# Autodesk Inventor assembly: Drive Roller Assembly 3 (Lexan)
(part 2 of 2)
- Mate:1223: Vex Pro End Bearing Mount (Bolt):1 ↔ Bearing Mount Spacer 1-8 in:1
- Mate:1224: Vex Pro 1x1 rectangular tubing 14 in length:5 ↔ Bearing Mount Spacer 1-8 in:2
- Mate:1225: Vex Pro 1x1 rectangular tubing 14 in length:5 ↔ Bearing Mount Spacer 1-8 in:2
- Mate:1226: Vex Pro 1x1 rectangular tubing 14 in length:5 ↔ Bearing Mount Spacer 1-8 in:2
- Mate:1227: Vex Pro End Bearing Mount (Bolt):2 ↔ Bearing Mount Spacer 1-8 in:2
- Mate:1228: Vex Pro End Bearing Mount (Bolt):2 ↔ Bearing Mount Spacer 1-8 in:2
- Mate:1229: Vex Pro End Bearing Mount (Bolt):2 ↔ Bearing Mount Spacer 1-8 in:2
- Mate:1230: Vex Pro 1x1 rectangular tubing 14 in length:6 ↔ Bearing Mount Spacer 1-8 in:3
- Mate:1231: Vex Pro 1x1 rectangular tubing 14 in length:6 ↔ Bearing Mount Spacer 1-8 in:3
- Mate:1232: Vex Pro 1x1 rectangular tubing 14 in length:6 ↔ Bearing Mount Spacer 1-8 in:3
- Mate:1233: Vex Pro End Bearing Mount (Bolt):3 ↔ Bearing Mount Spacer 1-8 in:3
- Mate:1234: Vex Pro End Bearing Mount (Bolt):3 ↔ Bearing Mount Spacer 1-8 in:3
- Mate:1235: Vex Pro End Bearing Mount (Bolt):3 ↔ Bearing Mount Spacer 1-8 in:3
- Mate:1236: Vex Pro 1x1 rectangular tubing 14 in length:6 ↔ Bearing Mount Spacer 1-8 in:5
- Mate:1237: Vex Pro 1x1 rectangular tubing 14 in length:6 ↔ Bearing Mount Spacer 1-8 in:5
- Mate:1238: Vex Pro 1x1 rectangular tubing 14 in length:6 ↔ Bearing Mount Spacer 1-8 in:5
- Mate:1239: Vex Pro End Bearing Mount (Bolt):4 ↔ Bearing Mount Spacer 1-8 in:5
- Mate:1240: Vex Pro End Bearing Mount (Bolt):4 ↔ Bearing Mount Spacer 1-8 in:5
- Mate:1241: Vex Pro End Bearing Mount (Bolt):4 ↔ Bearing Mount Spacer 1-8 in:5
- Mate:1242: Hex Shaft Collar 3-8 in (7552K300):1 ↔ Hex Shaft 3-8 in (am-0855):3
- Mate:1243: Hex Shaft Collar 3-8 in (7552K300):1 ↔ Hex Shaft 3-8 in (am-0855):3
- Flush:41: Hex Shaft Collar 3-8 in (7552K300):1 ↔ Hex Shaft 3-8 in (am-0855):3
- Mate:1244: Hex Shaft Collar 3-8 in (7552K300):3 ↔ Hex Shaft 3-8 in (am-0855):4
- Mate:1245: Hex Shaft Collar 3-8 in (7552K300):3 ↔ Hex Shaft 3-8 in (am-0855):4
- Flush:42: Hex Shaft Collar 3-8 in (7552K300):3 ↔ Hex Shaft 3-8 in (am-0855):4
- Mate:1246: Vex Pro 1x1 rectangular tubing 14 in length:5 ↔ Vex Pro T gusset - OUT OF STOCK 1192014:3
- Mate:1247: Vex Pro 1x1 rectangular tubing 14 in length:5 ↔ Vex Pro T gusset - OUT OF STOCK 1192014:3
- Mate:1248: Vex Pro 1x1 rectangular tubing 14 in length:5 ↔ Vex Pro T gusset - OUT OF STOCK 1192014:3
- Mate:1249: Vex Pro 1x1 rectangular tubing 4 in length:1 ↔ Vex Pro T gusset - OUT OF STOCK 1192014:3
- Mate:1250: Vex Pro 1x1 rectangular tubing 14 in length:5 ↔ Vex Pro T gusset - OUT OF STOCK 1192014:4
- Mate:1251: Vex Pro 1x1 rectangular tubing 14 in length:5 ↔ Vex Pro T gusset - OUT OF STOCK 1192014:4
- Mate:1252: Vex Pro 1x1 rectangular tubing 14 in length:5 ↔ Vex Pro T gusset - OUT OF STOCK 1192014:4
- Mate:1253: Vex Pro 1x1 rectangular tubing 4 in length:1 ↔ Vex Pro T gusset - OUT OF STOCK 1192014:4
- Mate:1254: Vex Pro 1x1 rectangular tubing 14 in length:6 ↔ Vex Pro T gusset - OUT OF STOCK 1192014:5
- Mate:1255: Vex Pro 1x1 rectangular tubing 14 in length:6 ↔ Vex Pro T gusset - OUT OF STOCK 1192014:5
- Mate:1256: Vex Pro 1x1 rectangular tubing 14 in length:6 ↔ Vex Pro T gusset - OUT OF STOCK 1192014:5
- Mate:1257: Vex Pro 1x1 rectangular tubing 4 in length:2 ↔ Vex Pro T gusset - OUT OF STOCK 1192014:5
- Mate:1258: Vex Pro 1x1 rectangular tubing 4 in length:1 ↔ Vex Pro T gusset - OUT OF STOCK 1192014:3
- Mate:1259: Vex Pro 1x1 rectangular tubing 4 in length:2 ↔ Vex Pro T gusset - OUT OF STOCK 1192014:5
- Mate:1260: Vex Pro 1x1 rectangular tubing 14 in length:6 ↔ Vex Pro T gusset - OUT OF STOCK 1192014:6
- Mate:1261: Vex Pro 1x1 rectangular tubing 14 in length:6 ↔ Vex Pro T gusset - OUT OF STOCK 1192014:6
- Mate:1262: Vex Pro 1x1 rectangular tubing 14 in length:6 ↔ Vex Pro T gusset - OUT OF STOCK 1192014:6
- Mate:1263: Vex Pro 1x1 rectangular tubing 4 in length:2 ↔ Vex Pro T gusset - OUT OF STOCK 1192014:6
- Mate:1264: Vex Pro 1x1 rectangular tubing 4 in length:2 ↔ Vex Pro T gusset - OUT OF STOCK 1192014:6
- Mate:1265: Vex Pro 1x1 rectangular tubing 4 in length:1 ↔ Vex Pro T gusset - OUT OF STOCK 1192014:3
## Named parameters: d240_d195 = 0 mm, d241_d196 = 0 mm, d242_d197 = 0 mm, d243_d198 = 0 mm, d305_d302 = 0 mm, d306_d303 = 0 mm, d307_d304 = 0 mm, d334_d317 = 0 mm, d339_d304 = 0 mm, d343_d308 = 0 mm, d344_d309 = 0 mm, d345_d310 = 0 mm, d346_d316 = 0 mm, d349_d328 = 0 mm, d350_d329 = 0 mm, d352_d331 = 0 mm, d353_d332 = 0 mm, d770_d743 = 0 mm, d771_d744 = 0 mm, d772_d745 = 0 mm, d773_d746 = 0 mm, d791_d742 = 0 mm, d1331_d1327 = 0 mm, d1332_d1328 = 0 mm, d1398_d1387 = 0 mm, d1399_d1388 = 0 mm, d1400_d1389 = 0 mm, d1404_d1384 = 0 mm, d1405_d1385 = 0 mm, d1406_d1386 = 0 mm
